# Autodesk Inventor assembly: POM_T5_03_nishio
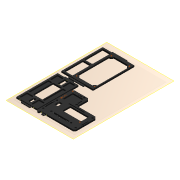
[picture p0: Inventor's stored thumbnail of the model, 180x180]
Saved by Autodesk Inventor 2022 (Build 260153000, 153)
## iProperties
Created: 2022-09-28
Part Number: POM_T5_03_nishio
Document SubType Name: Assembly
Designer: Masato
Author: Masato
## Documents named in this file (5)
- C:\Users\西尾　唯右吾\CITBrains\SUSTAINA-OP\Cam\POM_T5\POM_T5_03_nishio.iam
- C:\Users\西尾　唯右吾\CITBrains\SUSTAINA-OP\Cam\DisposableBoard.ipt
- C:\Users\西尾　唯右吾\CITBrains\SUSTAINA-OP\UpperBody\Cockpit\Cockpit_side_frame.ipt
- C:\Users\西尾　唯右吾\CITBrains\SUSTAINA-OP\UpperBody\Cockpit\Cockpit_circuit_board_frame.ipt
- C:\Users\西尾　唯右吾\CITBrains\SUSTAINA-OP\UpperBody\Cockpit\Cockpit_back_frame.ipt
## Components (4 placed, 4 different names)
1. DisposableBoard:1 — フラッシュ:1, フラッシュ:2, フラッシュ:3, フラッシュ:4, フラッシュ:5, フラッシュ:6, フラッシュ:8
2. Cockpit_side_frame:2 — メイト:3, メイト:4, フラッシュ:7
3. Cockpit_circuit_board_frame:1 — メイト:5, フラッシュ:8, メイト:6
4. Cockpit_back_frame:1 — メイト:1, フラッシュ:5, フラッシュ:6, メイト:4, フラッシュ:7, メイト:6
## Relationships (13: Flush 8, Mate 5)
- フラッシュ:1 [Flush]: DisposableBoard:1
- フラッシュ:2 [Flush]: DisposableBoard:1
- フラッシュ:3 [Flush]: DisposableBoard:1
- フラッシュ:4 [Flush]: DisposableBoard:1
- メイト:1 [Mate]: Cockpit_back_frame:1
- メイト:3 [Mate]: Cockpit_side_frame:2
- フラッシュ:5 [Flush] (2 mm): DisposableBoard:1 ↔ Cockpit_back_frame:1
- フラッシュ:6 [Flush] (2 mm): DisposableBoard:1 ↔ Cockpit_back_frame:1
- メイト:4 [Mate] (2.5 mm): Cockpit_side_frame:2 ↔ Cockpit_back_frame:1
- フラッシュ:7 [Flush]: Cockpit_side_frame:2 ↔ Cockpit_back_frame:1
- メイト:5 [Mate]: Cockpit_circuit_board_frame:1
- フラッシュ:8 [Flush] (2 mm): DisposableBoard:1 ↔ Cockpit_circuit_board_frame:1
- メイト:6 [Mate] (2.5 mm): Cockpit_circuit_board_frame:1 ↔ Cockpit_back_frame:1
